# Autodesk Inventor assembly: chwytak
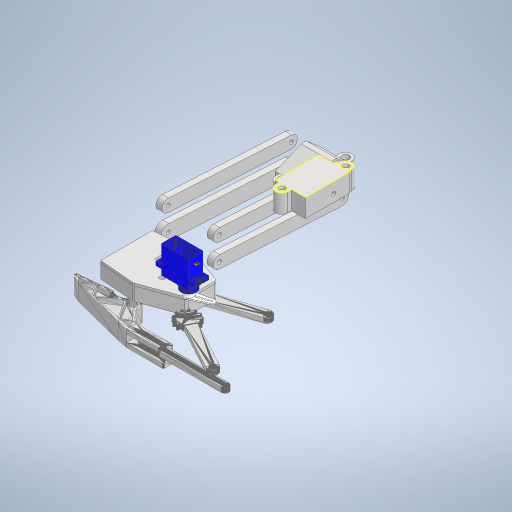
[picture p0: Inventor's stored thumbnail of the model, 512x512]
Saved by Autodesk Inventor 2023 (Build 270158000, 158)
## iProperties
Created: 2024-05-12
Part Number: chwytak
Document SubType Name: Assembly
Designer: kamil
Author: kamil
## Documents named in this file (12)
- C:\Users\kamil\Documents\PROJECTS - repos\ModBot---Projekt-Zespolowy\mechanics\modul_chwytaka\chwytak.iam
- C:\Users\kamil\Documents\PROJECTS - repos\ModBot---Projekt-Zespolowy\mechanics\modul_chwytaka\belka.ipt
- C:\Users\kamil\Documents\PROJECTS - repos\ModBot---Projekt-Zespolowy\mechanics\modul_chwytaka\Towerpro Micro Servo 9g.ipt
- C:\Users\kamil\Documents\PROJECTS - repos\ModBot---Projekt-Zespolowy\mechanics\modul_chwytaka\A1.ipt
- C:\Users\kamil\Documents\PROJECTS - repos\ModBot---Projekt-Zespolowy\mechanics\modul_chwytaka\uchwyt_serwa.ipt
- C:\Users\kamil\Documents\PROJECTS - repos\ModBot---Projekt-Zespolowy\mechanics\modul_chwytaka\belka_2.ipt
- C:\Users\kamil\Documents\PROJECTS - repos\ModBot---Projekt-Zespolowy\mechanics\modul_chwytaka\uchwyt_gorny.ipt
- C:\Users\kamil\Documents\PROJECTS - repos\ModBot---Projekt-Zespolowy\mechanics\modul_chwytaka\base_edited.ipt
- C:\Users\kamil\Documents\PROJECTS - repos\ModBot---Projekt-Zespolowy\mechanics\modul_chwytaka\Servo_Connector_Gear.ipt
- C:\Users\kamil\Documents\PROJECTS - repos\ModBot---Projekt-Zespolowy\mechanics\modul_chwytaka\Claw.ipt
- C:\Users\kamil\Documents\PROJECTS - repos\ModBot---Projekt-Zespolowy\mechanics\modul_chwytaka\Connector.ipt
- C:\Users\kamil\Documents\PROJECTS - repos\ModBot---Projekt-Zespolowy\mechanics\modul_chwytaka\Connector_Gear.ipt
## Components (15 placed, 11 different names)
1. belka:1 — Zestawiające:4, Zestawiające:5, Kątowe:1, Zestawiające:12, Równoległe:3
2. Towerpro Micro Servo 9g:1 — Zestawiające:1, Zestawiające:2, Równoległe:1, Zestawiające:3, Zestawiające:6, Zestawiające:7, Zestawiające:8, Zestawiające:9
3. A1:1 — Zestawiające:2, Zestawiające:3, Zestawiające:4, Zestawiające:5, Kątowe:1
4. uchwyt_serwa:1 — Zestawiające:7, Zestawiające:8, Zestawiające:9, Zestawiające:10, Zestawiające:11, Zestawiające:13, Zestawiające:14, Zestawiające:15
5. belka_2:1 — Zestawiające:10, Zestawiające:11, Zestawiające:12, Równoległe:2, Kątowe:2
6. uchwyt_gorny:1 — Zestawiające:13, Zestawiające:14, Zestawiające:15, Zestawiające:16, Zestawiające:17
7. belka_2:2 — Zestawiające:16, Równoległe:2, Kątowe:2, Równoległe:4
8. belka_2:3 — Zestawiające:17, Równoległe:3, Równoległe:4
9. base_edited:1 — Zestawiające:24, Zestawiające:25, Zestawiające:26
10. Servo_Connector_Gear:1 — Zestawiające:29, Zestawiające:30, Zestawiające:31
11. Claw:1
12. Connector:1
13. Connector_Gear:1
14. Towerpro Micro Servo 9g:2 — Zestawiające:24, Zestawiające:25, Zestawiające:26, Zestawiające:27, Zestawiające:28
15. A1:2 — Zestawiające:27, Zestawiające:28, Zestawiające:29, Zestawiające:30, Zestawiające:31
## Relationships (31: Mate 25, Flush 4, Angle 2)
- Zestawiające:1 [Mate]: Towerpro Micro Servo 9g:1
- Zestawiające:2 [Mate]: Towerpro Micro Servo 9g:1 ↔ A1:1
- Równoległe:1 [Flush]: Towerpro Micro Servo 9g:1
- Zestawiające:3 [Mate]: Towerpro Micro Servo 9g:1 ↔ A1:1
- Zestawiające:4 [Mate]: belka:1 ↔ A1:1
- Zestawiające:5 [Mate]: belka:1 ↔ A1:1
- Kątowe:1 [Angle] (180 deg): belka:1 ↔ A1:1
- Zestawiające:6 [Mate]: Towerpro Micro Servo 9g:1
- Zestawiające:7 [Mate]: Towerpro Micro Servo 9g:1 ↔ uchwyt_serwa:1
- Zestawiające:8 [Mate] (0.5 mm): Towerpro Micro Servo 9g:1 ↔ uchwyt_serwa:1
- Zestawiające:9 [Mate]: Towerpro Micro Servo 9g:1 ↔ uchwyt_serwa:1
- Zestawiające:10 [Mate] (2 mm): uchwyt_serwa:1 ↔ belka_2:1
- Zestawiające:11 [Mate]: uchwyt_serwa:1 ↔ belka_2:1
- Zestawiające:12 [Mate]: belka:1 ↔ belka_2:1
- Zestawiające:13 [Mate]: uchwyt_serwa:1 ↔ uchwyt_gorny:1
- Zestawiające:14 [Mate]: uchwyt_serwa:1 ↔ uchwyt_gorny:1
- Zestawiające:15 [Mate]: uchwyt_serwa:1 ↔ uchwyt_gorny:1
- Zestawiające:16 [Mate]: uchwyt_gorny:1 ↔ belka_2:2
- Równoległe:2 [Flush]: belka_2:1 ↔ belka_2:2
- Kątowe:2 [Angle] (180 deg): belka_2:1 ↔ belka_2:2
- Zestawiające:17 [Mate]: uchwyt_gorny:1 ↔ belka_2:3
- Równoległe:3 [Flush]: belka:1 ↔ belka_2:3
- Równoległe:4 [Flush]: belka_2:2 ↔ belka_2:3
- Zestawiające:24 [Mate] (0.3 mm): base_edited:1 ↔ Towerpro Micro Servo 9g:2
- Zestawiające:25 [Mate]: base_edited:1 ↔ Towerpro Micro Servo 9g:2
- Zestawiające:26 [Mate] (0.05 mm): base_edited:1 ↔ Towerpro Micro Servo 9g:2
- Zestawiające:27 [Mate]: Towerpro Micro Servo 9g:2 ↔ A1:2
- Zestawiające:28 [Mate]: Towerpro Micro Servo 9g:2 ↔ A1:2
- Zestawiające:29 [Mate]: Servo_Connector_Gear:1 ↔ A1:2
- Zestawiające:30 [Mate]: Servo_Connector_Gear:1 ↔ A1:2
- Zestawiające:31 [Mate]: Servo_Connector_Gear:1 ↔ A1:2
